# Autodesk Inventor assembly: Scrambler II
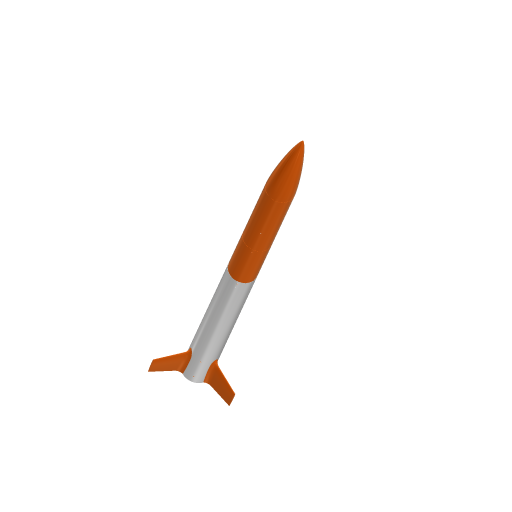
[picture p0: Inventor's stored thumbnail of the model, 512x512]
Saved by Autodesk Inventor 2024 (Build 280153000, 153)
## iProperties
Created: 2023-12-30
Part Number: Scrambler II
Document SubType Name: Assembly
Designer: Jamie
Mass: 631.455 g
Surface Area: 5625.65 cm^2
Volume: 391.502 cm^3
Density: 1.6129 g/cm^3
Author: Jamie
## Documents named in this file (5)
- C:\Users\Jamie\Documents\Uni\DARE\Scrambler-2-CAD\Autodesk\Scrambler II.iam
- C:\Users\Jamie\Documents\Uni\DARE\Scrambler-2-CAD\Autodesk\Structure.iam
- C:\Users\Jamie\Documents\Uni\DARE\Scrambler-2-CAD\Autodesk\Lower skin.ipt
- C:\Users\Jamie\Documents\Uni\DARE\Scrambler-2-CAD\Autodesk\Upper skin.ipt
- C:\Users\Jamie\Documents\Uni\DARE\Scrambler-2-CAD\Autodesk\Nosecone.ipt
## Components (4 placed, 4 different names)
1. Structure:1 [sub-assembly] — Mate:1, Mate:2, Mate:3, Mate:4, Mate:5, Angle:1
2. Lower skin:1 — Mate:1, Mate:2
3. Upper skin:1 — Mate:3, Mate:4, Mate:6
4. Nosecone:1 — Mate:5, Angle:1, Mate:6
## Relationships (7: Mate 6, Angle 1)
- Mate:1: Structure:1 ↔ Lower skin:1
- Mate:2: Structure:1 ↔ Lower skin:1
- Mate:3: Structure:1 ↔ Upper skin:1
- Mate:4: Structure:1 ↔ Upper skin:1
- Mate:5: Structure:1 ↔ Nosecone:1
- Angle:1 (12 deg): Structure:1 ↔ Nosecone:1
- Mate:6: Upper skin:1 ↔ Nosecone:1
